# Autodesk Inventor assembly: tssop
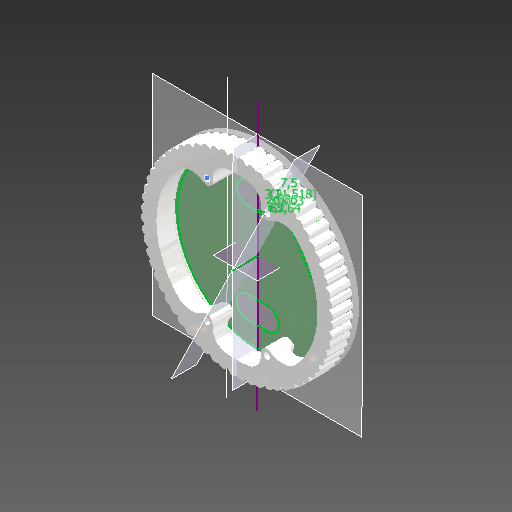
[picture p0: Inventor's stored thumbnail of the model, 512x512]
Saved by Autodesk Inventor 2023 (Build 270158000, 158)
## iProperties
Created: 2025-06-30
Part Number: tssop
Document SubType Name: Assembly
Designer: daa
Author: daa
## Documents named in this file (4)
- C:\Users\daa\Documents\DASH_V2\tssop.iam
- C:\Users\daa\Documents\DASH_\Dash-V1\кольцо.ipt
- C:\Users\daa\Documents\DASH_\Dash-V1\tssop3D\Board.iam
- C:\Users\daa\Documents\DASH_V2\tssopLid3.1.ipt
## Components (3 placed, 3 different names)
1. кольцо:1
2. Board:1 [sub-assembly] — С поворотом:1
3. tssopLid3.1:1 — С поворотом:1
## Relationships (1: RevoluteJoint 1)
- С поворотом:1 [RevoluteJoint]: Board:1 ↔ tssopLid3.1:1
